# Autodesk Inventor assembly: Schlitten
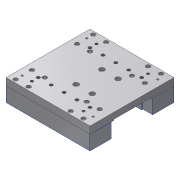
[picture p0: Inventor's stored thumbnail of the model, 180x180]
Saved by Autodesk Inventor 2016 (Build 200138000, 138)
## iProperties
Created: 2015-08-05
Part Number: Schlitten
Document SubType Name: Assembly
## Documents named in this file (6)
- E:\GitHub\CNC-Router_Z-Axis\Schlitten.iam
- E:\GitHub\CNC-Router_Z-Axis\Befestigungsplatte.ipt
- E:\GitHub\CNC-Router_Z-Axis\Distanzblock_rechts.ipt
- E:\GitHub\CNC-Router_Z-Axis\Distanzblock_links.ipt
- E:\GitHub\Standard-Parts\Schwerspannstift_ISO 8752 - 3 x 20_St-B.ipt
- E:\GitHub\Standard-Parts\Zyl-Schr_ISO 4762 - M5 x 25_St-Vzkt.ipt
## Components (11 placed, 5 different names)
1. Befestigungsplatte:1 — Flush:5, Flush:6, Flush:7, Mate:1, Mate:2, Insert:1, Insert:2, Insert:3, Insert:4
2. Distanzblock_rechts:1 — Mate:2, Insert:7, Insert:8
3. Distanzblock_links:1 — Mate:1, Insert:5, Insert:6
4. Schwerspannstift_ISO 8752 - 3 x 20_St-B:1 — Insert:1
5. Schwerspannstift_ISO 8752 - 3 x 20_St-B:2 — Insert:2
6. Schwerspannstift_ISO 8752 - 3 x 20_St-B:3 — Insert:3
7. Schwerspannstift_ISO 8752 - 3 x 20_St-B:4 — Insert:4
8. Zyl-Schr_ISO 4762 - M5 x 25_St-Vzkt:1 — Insert:5
9. Zyl-Schr_ISO 4762 - M5 x 25_St-Vzkt:2 — Insert:6
10. Zyl-Schr_ISO 4762 - M5 x 25_St-Vzkt:3 — Insert:7
11. Zyl-Schr_ISO 4762 - M5 x 25_St-Vzkt:4 — Insert:8
## Relationships (17: Insert 8, Flush 7, Mate 2)
- [Flush]: Befestigungsplatte:1 ↔ Distanzblock_links:1
- [Flush]: Befestigungsplatte:1 ↔ Distanzblock_links:1
- [Flush]: Befestigungsplatte:1 ↔ Distanzblock_rechts:1
- [Flush]: Befestigungsplatte:1 ↔ Distanzblock_rechts:1
- Flush:5: Befestigungsplatte:1
- Flush:6: Befestigungsplatte:1
- Flush:7: Befestigungsplatte:1
- Mate:1: Befestigungsplatte:1 ↔ Distanzblock_links:1
- Mate:2: Befestigungsplatte:1 ↔ Distanzblock_rechts:1
- Insert:1 (2 mm): Befestigungsplatte:1 ↔ Schwerspannstift_ISO 8752 - 3 x 20_St-B:1
- Insert:2 (2 mm): Befestigungsplatte:1 ↔ Schwerspannstift_ISO 8752 - 3 x 20_St-B:2
- Insert:3 (2 mm): Befestigungsplatte:1 ↔ Schwerspannstift_ISO 8752 - 3 x 20_St-B:3
- Insert:4 (2 mm): Befestigungsplatte:1 ↔ Schwerspannstift_ISO 8752 - 3 x 20_St-B:4
- Insert:5: Distanzblock_links:1 ↔ Zyl-Schr_ISO 4762 - M5 x 25_St-Vzkt:1
- Insert:6: Distanzblock_links:1 ↔ Zyl-Schr_ISO 4762 - M5 x 25_St-Vzkt:2
- Insert:7: Distanzblock_rechts:1 ↔ Zyl-Schr_ISO 4762 - M5 x 25_St-Vzkt:3
- Insert:8: Distanzblock_rechts:1 ↔ Zyl-Schr_ISO 4762 - M5 x 25_St-Vzkt:4
